# Autodesk Inventor assembly: First Stage
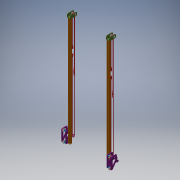
[picture p0: Inventor's stored thumbnail of the model, 180x180]
Saved by Autodesk Inventor 2017 SP1 (Build 210196100, 196)
## iProperties
Created: 2018-01-18
Part Number: First Stage
Document SubType Name: Assembly
Designer: Ben
Mass: 9979.66 g
Surface Area: 70095.8 cm^2
Volume: 103427 cm^3
Density: 0.0964899 g/cm^3
Author: Ben
## Documents named in this file (9)
- C:\Users\Ben\Desktop\Projects\2018 Robot\Cube Lift\First Stage.iam
- C:\Users\Ben\Desktop\Projects\2018 Robot\Cube Lift\Rail.ipt
- C:\Users\Ben\Desktop\Projects\2018 Robot\Cube Lift\roller bushing.iam
- C:\Users\Ben\Desktop\Projects\2018 Robot\Cube Lift\carriage plate square 2.ipt
- C:\Users\Ben\Desktop\Projects\2018 Robot\Cube Lift\top pully bracket 2.ipt
- C:\Users\Ben\Desktop\Projects\2018 Robot\Cube Lift\second stage belt 2.ipt
- C:\Users\Ben\Desktop\Projects\2018 Robot\Cube Lift\line pulley.ipt
- C:\Users\Ben\Desktop\Projects\2018 Robot\Cube Lift\outside carriage plate.ipt
- C:\Users\Ben\Desktop\Projects\2018 Robot\Cube Lift\first stage spacer.ipt
## Components (26 placed, 8 different names)
1. Rail:3 — Mate:5, Mate:24, Flush:34, Mate:48, Flush:35, Angle:4, Flush:64, Mate:104
2. roller bushing:1 [sub-assembly] — Mate:38, Insert:36
3. carriage plate square 2:1 — Mate:5, Mate:24, Mate:36, Mate:37, Mate:38, Mate:66, Mate:67, Mate:73, Mate:74, Mate:104
4. roller bushing:2 [sub-assembly] — Mate:36, Insert:34
5. roller bushing:3 [sub-assembly] — Mate:37, Insert:35
6. top pully bracket 2:1 — Flush:34, Mate:48, Flush:35, Mate:70, Mate:71
7. second stage belt 2:1 — Angle:4, Mate:68, Mate:69, Flush:66
8. line pulley:1 — Mate:66, Mate:67, Mate:68, Mate:69
9. line pulley:2 — Mate:70, Mate:71
10. outside carriage plate:1 — Mate:73, Mate:74
11. Rail:4 — Mate:86, Flush:58, Flush:59, Mate:93, Flush:60, Flush:64, Mate:103
12. outside carriage plate:2 — Insert:19, Insert:20, Insert:21, Mate:84, Mate:85
13. carriage plate square 2:2 — Mate:84, Mate:85, Mate:86, Flush:58, Insert:26, Mate:103
14. roller bushing:7 [sub-assembly] — Insert:19, Insert:32
15. roller bushing:8 [sub-assembly] — Insert:20, Insert:33
16. roller bushing:10 [sub-assembly] — Insert:21, Insert:31
17. line pulley:3 — Insert:26, Mate:101, Mate:102
18. top pully bracket 2:2 — Flush:59, Mate:93, Flush:60, Mate:97, Mate:98
19. line pulley:4 — Mate:97, Mate:98
20. second stage belt 2:2 — Mate:101, Mate:102, Flush:66
21. first stage spacer:1 — Insert:31
22. first stage spacer:2 — Insert:32
23. first stage spacer:3 — Insert:33
24. first stage spacer:4 — Insert:35
25. first stage spacer:5 — Insert:36
26. first stage spacer:6 — Insert:34
## Relationships (42: Mate 24, Insert 10, Flush 7, Angle 1)
- Mate:5: Rail:3 ↔ carriage plate square 2:1
- Mate:24: Rail:3 ↔ carriage plate square 2:1
- Mate:36: carriage plate square 2:1 ↔ roller bushing:2
- Mate:37: carriage plate square 2:1 ↔ roller bushing:3
- Mate:38: roller bushing:1 ↔ carriage plate square 2:1
- Flush:34 (-1.5875 mm): Rail:3 ↔ top pully bracket 2:1
- Mate:48: Rail:3 ↔ top pully bracket 2:1
- Flush:35 (-6.35 mm): Rail:3 ↔ top pully bracket 2:1
- Angle:4 (0 deg): Rail:3 ↔ second stage belt 2:1
- Mate:66: carriage plate square 2:1 ↔ line pulley:1
- Mate:67 (3.175 mm): carriage plate square 2:1 ↔ line pulley:1
- Mate:68: second stage belt 2:1 ↔ line pulley:1
- Mate:69 (0.7937 mm): second stage belt 2:1 ↔ line pulley:1
- Mate:70: top pully bracket 2:1 ↔ line pulley:2
- Mate:71 (4.7625 mm): top pully bracket 2:1 ↔ line pulley:2
- Mate:73: carriage plate square 2:1 ↔ outside carriage plate:1
- Mate:74: carriage plate square 2:1 ↔ outside carriage plate:1
- Insert:19: outside carriage plate:2 ↔ roller bushing:7
- Insert:20: outside carriage plate:2 ↔ roller bushing:8
- Insert:21: outside carriage plate:2 ↔ roller bushing:10
- Mate:84: outside carriage plate:2 ↔ carriage plate square 2:2
- Mate:85: outside carriage plate:2 ↔ carriage plate square 2:2
- Mate:86: Rail:4 ↔ carriage plate square 2:2
- Flush:58: Rail:4 ↔ carriage plate square 2:2
- Insert:26 (3.175 mm): carriage plate square 2:2 ↔ line pulley:3
- Flush:59 (1.5875 mm): Rail:4 ↔ top pully bracket 2:2
- Mate:93: Rail:4 ↔ top pully bracket 2:2
- Flush:60 (6.35 mm): Rail:4 ↔ top pully bracket 2:2
- Mate:97: top pully bracket 2:2 ↔ line pulley:4
- Mate:98 (4.7625 mm): top pully bracket 2:2 ↔ line pulley:4
- Flush:64: Rail:3 ↔ Rail:4
- Mate:101: line pulley:3 ↔ second stage belt 2:2
- Mate:102 (0.7937 mm): line pulley:3 ↔ second stage belt 2:2
- Flush:66: second stage belt 2:1 ↔ second stage belt 2:2
- Insert:31: roller bushing:10 ↔ first stage spacer:1
- Insert:32: roller bushing:7 ↔ first stage spacer:2
- Insert:33: roller bushing:8 ↔ first stage spacer:3
- Insert:34: roller bushing:2 ↔ first stage spacer:6
- Insert:35: roller bushing:3 ↔ first stage spacer:4
- Insert:36: roller bushing:1 ↔ first stage spacer:5
- Mate:103 (-12.7 mm): Rail:4 ↔ carriage plate square 2:2
- Mate:104 (-12.7 mm): Rail:3 ↔ carriage plate square 2:1
